# Autodesk Inventor assembly: ABI_Baugruppe
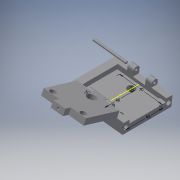
[picture p0: Inventor's stored thumbnail of the model, 180x180]
Saved by Autodesk Inventor 2018 (Build 220112000, 112)
## iProperties
Created: 2019-11-22
Part Number: ABI_Baugruppe
Material: Generisch
Document SubType Name: Assembly
Designer: Dubsky
Author: Dubsky
## Documents named in this file (9)
- C:\Users\Dubsky\Downloads\Biegevorrichtung\Daten\ABI_Baugruppe.iam
- C:\Users\Dubsky\Downloads\Biegevorrichtung\Daten\ABI_Arretierstift.ipt
- C:\Users\Dubsky\Downloads\Biegevorrichtung\Daten\ABI_Führungsblock.ipt
- C:\Users\Dubsky\Downloads\Biegevorrichtung\Daten\ABI_Grundplatte.ipt
- C:\Users\Dubsky\Downloads\Biegevorrichtung\Daten\ABI_Anschlag.ipt
- C:\Users\Dubsky\Downloads\Biegevorrichtung\Daten\ABI_Auswurf.ipt
- C:\Users\Dubsky\Downloads\Biegevorrichtung\Daten\ABI_Lagerbock.ipt
- C:\Users\Dubsky\Downloads\Biegevorrichtung\Daten\ABI_Stift.ipt
- C:\Users\Dubsky\Downloads\Biegevorrichtung\Daten\ABI_Deckel.ipt
## Components (8 placed, 8 different names)
1. ABI_Arretierstift:1 — Passend:12, Passend:13
2. ABI_Führungsblock:1 — Passend:1, Passend:3, Passend:10, Passend:11, Passend:14, Passend:15, Passend:16
3. ABI_Grundplatte:1 — Passend:1, Passend:2, Passend:3, Passend:4, Passend:5, Passend:6, Passend:8
4. ABI_Kasten:1 — Passend:6, Passend:7, Passend:16
5. ABI_Auswurf:1 — Passend:8, Passend:9, Passend:15
6. ABI_Lagerbock:1 — Passend:2, Passend:4, Passend:5, Passend:7, Passend:9, Passend:12, Passend:13
7. ABI_Stift:1 — Passend:11
8. ABI_Deckel:1 — Passend:10, Passend:14
## Relationships (16: Mate 16)
- Passend:1 [Mate]: ABI_Führungsblock:1 ↔ ABI_Grundplatte:1
- Passend:2 [Mate]: ABI_Grundplatte:1 ↔ ABI_Lagerbock:1
- Passend:3 [Mate]: ABI_Führungsblock:1 ↔ ABI_Grundplatte:1
- Passend:4 [Mate]: ABI_Grundplatte:1 ↔ ABI_Lagerbock:1
- Passend:5 [Mate]: ABI_Grundplatte:1 ↔ ABI_Lagerbock:1
- Passend:6 [Mate]: ABI_Grundplatte:1 ↔ ABI_Kasten:1
- Passend:7 [Mate]: ABI_Kasten:1 ↔ ABI_Lagerbock:1
- Passend:8 [Mate]: ABI_Grundplatte:1 ↔ ABI_Auswurf:1
- Passend:9 [Mate]: ABI_Auswurf:1 ↔ ABI_Lagerbock:1
- Passend:10 [Mate]: ABI_Führungsblock:1 ↔ ABI_Deckel:1
- Passend:11 [Mate]: ABI_Führungsblock:1 ↔ ABI_Stift:1
- Passend:12 [Mate]: ABI_Arretierstift:1 ↔ ABI_Lagerbock:1
- Passend:13 [Mate]: ABI_Arretierstift:1 ↔ ABI_Lagerbock:1
- Passend:14 [Mate]: ABI_Führungsblock:1 ↔ ABI_Deckel:1
- Passend:15 [Mate]: ABI_Führungsblock:1 ↔ ABI_Auswurf:1
- Passend:16 [Mate]: ABI_Führungsblock:1 ↔ ABI_Kasten:1
